# Autodesk Inventor assembly: Manipulator
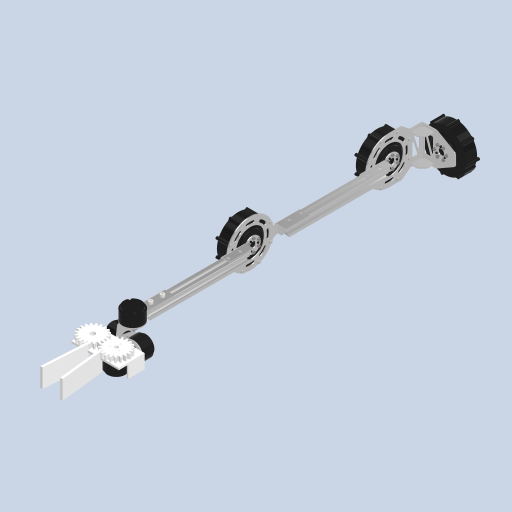
[picture p0: Inventor's stored thumbnail of the model, 512x512]
Saved by Autodesk Inventor 2023 (Build 270158000, 158)
## iProperties
Created: 2024-11-08
Part Number: Manipulator
Document SubType Name: Assembly
Designer: kiyo
Author: kiyo
## Documents named in this file (21)
- D:\GitHub\inventor\syu-si\OfficeRobot\Manipulator\Manipulator.iam
- D:\GitHub\inventor\syu-si\OfficeRobot\ReadyMade\Steadywin\GIM8108-8.iam
- D:\GitHub\inventor\syu-si\OfficeRobot\Manipulator\sholder-roll-bracket.ipt
- D:\GitHub\inventor\syu-si\OfficeRobot\Manipulator\elbow-pitch-bracket.ipt
- D:\GitHub\inventor\syu-si\OfficeRobot\Manipulator\Hand.iam
- D:\GitHub\inventor\syu-si\OfficeRobot\ReadyMade\Screw\M3_6mm.ipt
- D:\GitHub\inventor\syu-si\OfficeRobot\ReadyMade\Steadywin\GIM3505-8_with-driver.ipt
- D:\GitHub\inventor\syu-si\OfficeRobot\Manipulator\wrist_roll_plate.ipt
- D:\GitHub\inventor\syu-si\OfficeRobot\Manipulator\wrist-pitch-plate.ipt
- D:\GitHub\inventor\syu-si\OfficeRobot\Manipulator\wrist-yaw-plate.ipt
- D:\GitHub\inventor\syu-si\OfficeRobot\ReadyMade\Screw\M2-5_6mm.ipt
- D:\GitHub\inventor\syu-si\OfficeRobot\ReadyMade\Screw\SLBNR5.ipt
- D:\GitHub\inventor\syu-si\OfficeRobot\ReadyMade\Screw\CBSH3-8.ipt
- D:\GitHub\inventor\syu-si\OfficeRobot\ReadyMade\Screw\HNTT5-5.ipt
- D:\GitHub\inventor\syu-si\OfficeRobot\ReadyMade\Screw\SCB5-8.ipt
- D:\GitHub\inventor\syu-si\OfficeRobot\ReadyMade\Screw\FWSJJ-D5-V2_6-T4_5.ipt
- D:\GitHub\inventor\syu-si\OfficeRobot\ReadyMade\Screw\M2-5_10mm.ipt
- D:\GitHub\inventor\syu-si\OfficeRobot\ReadyMade\Screw\HNTU5-5.ipt
- D:\GitHub\inventor\syu-si\OfficeRobot\Manipulator\pitch_plate_20mm_kari.ipt
- D:\GitHub\inventor\syu-si\OfficeRobot\ReadyMade\Aluminum-frame\HFS5-2020-210-AV10-BV35-CV175-DV200.ipt
- D:\GitHub\inventor\syu-si\OfficeRobot\Manipulator\pitch_plate_20mm.ipt
## Components (88 placed, 20 different names)
1. sholder-roll-bracket:1 — 挿入:312, 挿入:313, 挿入:314, 角度:22
2. wrist_roll_plate:1 — 挿入:220, 挿入:227, 挿入:228, 挿入:229, 挿入:230, 挿入:231, 挿入:283, 挿入:284, 挿入:285
3. wrist-pitch-plate:1 — 挿入:211, 挿入:212, 挿入:213, 挿入:217, 挿入:218, 挿入:219, 挿入:220, 挿入:280, 挿入:281, 挿入:282
4. wrist-yaw-plate:1 — 挿入:203, 挿入:204, 挿入:205, 挿入:206, 挿入:207, 挿入:211, 挿入:258, 挿入:259, 挿入:291, 挿入:292, 挿入:346, 挿入:347
5. Hand:1 [sub-assembly] — ハンド, 挿入:301
6. SLBNR5:7 — 挿入:258
7. SLBNR5:8 — 挿入:259
8. FWSJJ-D5-V2_6-T4_5:7 — 挿入:286
9. FWSJJ-D5-V2_6-T4_5:8 — 挿入:287
10. FWSJJ-D5-V2_6-T4_5:9 — 挿入:288
11. HNTT5-5:3
12. HNTT5-5:4
13. SCB5-8:3 — 挿入:291
14. SCB5-8:4 — 挿入:292
15. HFS5-2020-210-AV10-BV35-CV175-DV200:1
16. HFS5-2020-210-AV10-BV35-CV175-DV200:2 — 挿入:346, 挿入:347
17. HNTU5-5:1
18. HNTU5-5:3
19. HNTU5-5:4
20. HNTU5-5:6
21. HNTU5-5:7
22. HNTU5-5:8
23. pitch_plate_20mm:1
24. elbow-pitch-bracket:1 — 挿入:341, 挿入:342
25. HNTU5-5:9
26. HNTU5-5:10
27. pitch_plate_20mm_kari:2 — 挿入:345, 角度:26
28. M3_6mm:1
29. M3_6mm:2
30. M3_6mm:3
31. M3_6mm:4
32. M3_6mm:5
33. M3_6mm:6
34. M3_6mm:7 — 挿入:337
35. M3_6mm:8 — 挿入:336
36. M3_6mm:9 — 挿入:334
37. M3_6mm:10 — 挿入:338
38. M3_6mm:11 — 挿入:339
39. M3_6mm:12 — 挿入:335
40. M3_6mm:13
41. M3_6mm:14
42. M3_6mm:15
43. M3_6mm:16
44. M3_6mm:17
45. M3_6mm:18
46. CBSH3-8:1 — 挿入:307
47. CBSH3-8:2 — 挿入:308
48. CBSH3-8:3 — 挿入:302
49. CBSH3-8:4 — 挿入:304
50. CBSH3-8:5 — 挿入:309
51. CBSH3-8:6 — 挿入:303
52. CBSH3-8:7 — 挿入:305
53. CBSH3-8:8 — 挿入:306
54. CBSH3-8:9 — 挿入:332
55. CBSH3-8:10 — 挿入:327
56. CBSH3-8:11 — 挿入:330
57. CBSH3-8:12 — 挿入:328
58. CBSH3-8:13 — 挿入:329
59. CBSH3-8:14 — 挿入:331
60. CBSH3-8:15 — 挿入:326
61. CBSH3-8:16 — 挿入:333
62. M2-5_6mm:1 — 挿入:205
63. M2-5_6mm:2 — 挿入:207
64. M2-5_6mm:3 — 挿入:206
65. M2-5_6mm:7 — 挿入:229
66. M2-5_6mm:8 — 挿入:230
67. M2-5_6mm:9 — 挿入:231
68. M2-5_6mm:4 — 挿入:217
69. M2-5_6mm:5 — 挿入:218
70. M2-5_6mm:6 — 挿入:219
71. M2-5_10mm:1
72. M2-5_10mm:2
73. M2-5_10mm:3
74. M2-5_10mm:4
75. M2-5_10mm:5
76. M2-5_10mm:6
77. FWSJJ-D5-V2_6-T4_5:1 — 挿入:280
78. FWSJJ-D5-V2_6-T4_5:2 — 挿入:282
79. FWSJJ-D5-V2_6-T4_5:3 — 挿入:281
80. FWSJJ-D5-V2_6-T4_5:4 — 挿入:283
81. FWSJJ-D5-V2_6-T4_5:5 — 挿入:285
82. FWSJJ-D5-V2_6-T4_5:6 — 挿入:284
83. GIM3505-8_with-driver:1 — 挿入:203, 挿入:204
84. GIM3505-8_with-driver:3 — 挿入:227, 挿入:228, 挿入:286, 挿入:287, 挿入:288, 挿入:301
85. GIM3505-8_with-driver:4 — 挿入:212, 挿入:213
86. GIM8108-8:1 [sub-assembly] — 挿入:312
87. GIM8108-8:2 [sub-assembly] — 挿入:302, 挿入:303, 挿入:304, 挿入:305, 挿入:306, 挿入:307, 挿入:308, 挿入:309, 挿入:313, 挿入:314
88. GIM8108-8:3 [sub-assembly] — 挿入:326, 挿入:327, 挿入:328, 挿入:329, 挿入:330, 挿入:331, 挿入:332, 挿入:333, 挿入:334, 挿入:335, 挿入:336, 挿入:337, 挿入:338, 挿入:339, 挿入:341, 挿入:342, 挿入:345
## Relationships (98: Insert 78, Angle 11, Mate 9)
- ハンド [Angle] (0 deg): Hand:1
- 挿入:203 [Insert]: wrist-yaw-plate:1 ↔ GIM3505-8_with-driver:1
- 挿入:204 [Insert]: wrist-yaw-plate:1 ↔ GIM3505-8_with-driver:1
- 挿入:205 [Insert]: wrist-yaw-plate:1 ↔ M2-5_6mm:1
- 挿入:206 [Insert]: wrist-yaw-plate:1 ↔ M2-5_6mm:3
- 挿入:207 [Insert]: wrist-yaw-plate:1 ↔ M2-5_6mm:2
- 挿入:211 [Insert] (3.5 mm): wrist-pitch-plate:1 ↔ wrist-yaw-plate:1
- 挿入:212 [Insert]: wrist-pitch-plate:1 ↔ GIM3505-8_with-driver:4
- 挿入:213 [Insert]: wrist-pitch-plate:1 ↔ GIM3505-8_with-driver:4
- 挿入:217 [Insert]: wrist-pitch-plate:1 ↔ M2-5_6mm:4
- 挿入:218 [Insert]: wrist-pitch-plate:1 ↔ M2-5_6mm:5
- 挿入:219 [Insert]: wrist-pitch-plate:1 ↔ M2-5_6mm:6
- 挿入:220 [Insert] (3.5 mm): wrist_roll_plate:1 ↔ wrist-pitch-plate:1
- [Insert]: wrist-pitch-plate:1 ↔ M2-5_10mm:1
- [Insert]: wrist-pitch-plate:1 ↔ M2-5_10mm:2
- [Insert]: wrist-pitch-plate:1 ↔ M2-5_10mm:3
- [Insert]: wrist_roll_plate:1 ↔ M2-5_10mm:6
- [Insert]: wrist_roll_plate:1 ↔ M2-5_10mm:4
- [Insert]: wrist_roll_plate:1 ↔ M2-5_10mm:5
- 挿入:227 [Insert]: wrist_roll_plate:1 ↔ GIM3505-8_with-driver:3
- 挿入:228 [Insert]: wrist_roll_plate:1 ↔ GIM3505-8_with-driver:3
- 挿入:229 [Insert]: wrist_roll_plate:1 ↔ M2-5_6mm:7
- 挿入:230 [Insert]: wrist_roll_plate:1 ↔ M2-5_6mm:8
- 挿入:231 [Insert]: wrist_roll_plate:1 ↔ M2-5_6mm:9
- 挿入:258 [Insert]: wrist-yaw-plate:1 ↔ SLBNR5:7
- 挿入:259 [Insert]: wrist-yaw-plate:1 ↔ SLBNR5:8
- 挿入:280 [Insert]: wrist-pitch-plate:1 ↔ FWSJJ-D5-V2_6-T4_5:1
- 挿入:281 [Insert]: wrist-pitch-plate:1 ↔ FWSJJ-D5-V2_6-T4_5:3
- 挿入:282 [Insert]: wrist-pitch-plate:1 ↔ FWSJJ-D5-V2_6-T4_5:2
- 挿入:283 [Insert]: wrist_roll_plate:1 ↔ FWSJJ-D5-V2_6-T4_5:4
- 挿入:284 [Insert]: wrist_roll_plate:1 ↔ FWSJJ-D5-V2_6-T4_5:6
- 挿入:285 [Insert]: wrist_roll_plate:1 ↔ FWSJJ-D5-V2_6-T4_5:5
- 挿入:286 [Insert]: FWSJJ-D5-V2_6-T4_5:7 ↔ GIM3505-8_with-driver:3
- 挿入:287 [Insert]: FWSJJ-D5-V2_6-T4_5:8 ↔ GIM3505-8_with-driver:3
- 挿入:288 [Insert]: FWSJJ-D5-V2_6-T4_5:9 ↔ GIM3505-8_with-driver:3
- [Insert] (3.2 mm): HNTT5-5:3 ↔ SCB5-8:3
- [Insert] (3.2 mm): HNTT5-5:4 ↔ SCB5-8:4
- 挿入:291 [Insert]: wrist-yaw-plate:1 ↔ SCB5-8:3
- 挿入:292 [Insert]: wrist-yaw-plate:1 ↔ SCB5-8:4
- 挿入:301 [Insert] (4.5 mm): Hand:1 ↔ GIM3505-8_with-driver:3
- 挿入:302 [Insert] (2 mm): CBSH3-8:3 ↔ GIM8108-8:2
- 挿入:303 [Insert] (2 mm): CBSH3-8:6 ↔ GIM8108-8:2
- 挿入:304 [Insert] (2 mm): CBSH3-8:4 ↔ GIM8108-8:2
- 挿入:305 [Insert] (2 mm): CBSH3-8:7 ↔ GIM8108-8:2
- 挿入:306 [Insert] (2 mm): CBSH3-8:8 ↔ GIM8108-8:2
- 挿入:307 [Insert] (2 mm): CBSH3-8:1 ↔ GIM8108-8:2
- 挿入:308 [Insert] (2 mm): CBSH3-8:2 ↔ GIM8108-8:2
- 挿入:309 [Insert] (2 mm): CBSH3-8:5 ↔ GIM8108-8:2
- 挿入:312 [Insert]: sholder-roll-bracket:1 ↔ GIM8108-8:1
- 挿入:313 [Insert]: sholder-roll-bracket:1 ↔ GIM8108-8:2
- 挿入:314 [Insert]: sholder-roll-bracket:1 ↔ GIM8108-8:2
- [Insert] (-0.75 mm): HFS5-2020-210-AV10-BV35-CV175-DV200:2 ↔ HNTU5-5:1
- [Insert] (-0.75 mm): HFS5-2020-210-AV10-BV35-CV175-DV200:2 ↔ HNTU5-5:4
- [Insert] (-0.75 mm): HFS5-2020-210-AV10-BV35-CV175-DV200:2 ↔ HNTU5-5:3
- [Insert] (-0.75 mm): HFS5-2020-210-AV10-BV35-CV175-DV200:2 ↔ HNTU5-5:8
- [Angle] (0 deg): HFS5-2020-210-AV10-BV35-CV175-DV200:2 ↔ HNTU5-5:1
- [Angle] (0 deg): HFS5-2020-210-AV10-BV35-CV175-DV200:2 ↔ HNTU5-5:4
- [Insert] (-0.75 mm): HFS5-2020-210-AV10-BV35-CV175-DV200:1 ↔ HNTU5-5:6
- [Angle] (0 deg): HFS5-2020-210-AV10-BV35-CV175-DV200:1 ↔ HNTU5-5:6
- [Insert] (-0.75 mm): HFS5-2020-210-AV10-BV35-CV175-DV200:1 ↔ HNTU5-5:7
- [Angle] (0 deg): HFS5-2020-210-AV10-BV35-CV175-DV200:1 ↔ HNTU5-5:7
- [Angle] (0 deg): HFS5-2020-210-AV10-BV35-CV175-DV200:1 ↔ HNTU5-5:6
- 角度:22 [Angle] (0 deg): sholder-roll-bracket:1
- 挿入:326 [Insert] (2 mm): CBSH3-8:15 ↔ GIM8108-8:3
- 挿入:327 [Insert] (2 mm): CBSH3-8:10 ↔ GIM8108-8:3
- 挿入:328 [Insert] (2 mm): CBSH3-8:12 ↔ GIM8108-8:3
- 挿入:329 [Insert] (2 mm): CBSH3-8:13 ↔ GIM8108-8:3
- 挿入:330 [Insert] (2 mm): CBSH3-8:11 ↔ GIM8108-8:3
- 挿入:331 [Insert] (2 mm): CBSH3-8:14 ↔ GIM8108-8:3
- 挿入:332 [Insert] (2 mm): CBSH3-8:9 ↔ GIM8108-8:3
- 挿入:333 [Insert] (2 mm): CBSH3-8:16 ↔ GIM8108-8:3
- 挿入:334 [Insert] (2 mm): M3_6mm:9 ↔ GIM8108-8:3
- 挿入:335 [Insert] (2 mm): M3_6mm:12 ↔ GIM8108-8:3
- 挿入:336 [Insert] (2 mm): M3_6mm:8 ↔ GIM8108-8:3
- 挿入:337 [Insert] (2 mm): M3_6mm:7 ↔ GIM8108-8:3
- 挿入:338 [Insert] (2 mm): M3_6mm:10 ↔ GIM8108-8:3
- 挿入:339 [Insert] (2 mm): M3_6mm:11 ↔ GIM8108-8:3
- [Insert]: pitch_plate_20mm:1 ↔ GIM8108-8:2
- [Mate] (4 mm): HFS5-2020-210-AV10-BV35-CV175-DV200:1 ↔ pitch_plate_20mm:1
- [Mate]: HFS5-2020-210-AV10-BV35-CV175-DV200:1 ↔ pitch_plate_20mm:1
- [Mate]: HFS5-2020-210-AV10-BV35-CV175-DV200:1 ↔ pitch_plate_20mm:1
- 挿入:341 [Insert]: elbow-pitch-bracket:1 ↔ GIM8108-8:3
- 挿入:342 [Insert]: elbow-pitch-bracket:1 ↔ GIM8108-8:3
- [Angle] (0 deg): HFS5-2020-210-AV10-BV35-CV175-DV200:1 ↔ HNTU5-5:9
- [Angle] (0 deg): HFS5-2020-210-AV10-BV35-CV175-DV200:1 ↔ HNTU5-5:10
- [Insert] (-0.75 mm): HFS5-2020-210-AV10-BV35-CV175-DV200:1 ↔ HNTU5-5:9
- [Insert] (-0.75 mm): HFS5-2020-210-AV10-BV35-CV175-DV200:1 ↔ HNTU5-5:10
- [Mate]: HFS5-2020-210-AV10-BV35-CV175-DV200:1 ↔ elbow-pitch-bracket:1
- [Mate] (4 mm): HFS5-2020-210-AV10-BV35-CV175-DV200:1 ↔ elbow-pitch-bracket:1
- [Mate]: HFS5-2020-210-AV10-BV35-CV175-DV200:1 ↔ elbow-pitch-bracket:1
- [Angle] (0 deg): pitch_plate_20mm:1
- 挿入:345 [Insert]: pitch_plate_20mm_kari:2 ↔ GIM8108-8:3
- [Mate]: HFS5-2020-210-AV10-BV35-CV175-DV200:2 ↔ pitch_plate_20mm_kari:2
- [Mate]: HFS5-2020-210-AV10-BV35-CV175-DV200:2 ↔ pitch_plate_20mm_kari:2
- [Mate] (4 mm): HFS5-2020-210-AV10-BV35-CV175-DV200:2 ↔ pitch_plate_20mm_kari:2
- 挿入:346 [Insert]: wrist-yaw-plate:1 ↔ HFS5-2020-210-AV10-BV35-CV175-DV200:2
- 挿入:347 [Insert]: wrist-yaw-plate:1 ↔ HFS5-2020-210-AV10-BV35-CV175-DV200:2
- 角度:26 [Angle] (0 deg): pitch_plate_20mm_kari:2
## Named parameters: d332_d317 = 3.2 mm, d333_d318 = 3.2 mm
